# Autodesk Inventor assembly: v5马达-01
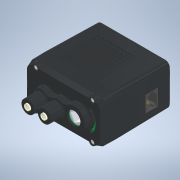
[picture p0: Inventor's stored thumbnail of the model, 180x180]
Saved by Autodesk Inventor 2020 (Build 240168000, 168)
## iProperties
Created: 2019-06-06
Part Number: v5马达-01
Document SubType Name: Assembly
Designer: aresp
Author: aresp
## Documents named in this file (8)
- D:\vault\ncrCadLib\V5主控系统\v5马达.iam
- D:\vault\ncrCadLib\V5主控系统\v5马达.ipt
- C:\Users\aresp\Documents\Inventor\Content Center Files\R2020\zh-CN\Screw 8-32 x 0.500'' 三号\275-1004-001.ipt
- C:\Users\aresp\Documents\Inventor\Content Center Files\R2020\zh-CN\细轴四方轴承\常规.ipt
- C:\Users\aresp\Documents\Inventor\Content Center Files\R2020\zh-CN\Screw 8-32 x 0.625'' 四号\275-1005-001.ipt
- v5马达.iam
- v5马达+螺丝.iam
- v5马达+螺丝+轴承.iam
## Components (6 placed, 4 different names)
1. v5马达:1 — 配合:3, 配合:8, 配合:9
2. 细轴四方轴承 常规:1 — 配合:3, 配合:4, 配合:5, 配合:6
3. Screw 8-32 x 0.500'' 三号 275-1004-001:1 — 配合:4, 配合:7
4. Screw 8-32 x 0.500'' 三号 275-1004-001:2 — 配合:5, 配合:8, 配合:9
5. Screw 8-32 x 0.625'' 四号 275-1005-001:1 — 配合:6, 配合:7
6. Screw 8-32 x 0.625'' 四号 275-1005-001:2
## Component patterns: (2 elements, first: Screw 8-32 x 0.500'' 三号 275-1004-001:1), (2 elements, first: Screw 8-32 x 0.625'' 四号 275-1005-001:1)
## Relationships (7: Mate 7)
- 配合:3 [Mate] (1.5748 mm): v5马达:1 ↔ 细轴四方轴承 常规:1
- 配合:4 [Mate]: 细轴四方轴承 常规:1 ↔ Screw 8-32 x 0.500'' 三号 275-1004-001:1
- 配合:5 [Mate]: 细轴四方轴承 常规:1 ↔ Screw 8-32 x 0.500'' 三号 275-1004-001:2
- 配合:6 [Mate]: 细轴四方轴承 常规:1 ↔ Screw 8-32 x 0.625'' 四号 275-1005-001:1
- 配合:7 [Mate]: Screw 8-32 x 0.500'' 三号 275-1004-001:1 ↔ Screw 8-32 x 0.625'' 四号 275-1005-001:1
- 配合:8 [Mate] (1.5748 mm): v5马达:1 ↔ Screw 8-32 x 0.500'' 三号 275-1004-001:2
- 配合:9 [Mate]: v5马达:1 ↔ Screw 8-32 x 0.500'' 三号 275-1004-001:2
